# Autodesk Inventor assembly: Sensor_Test
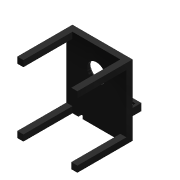
[picture p0: Inventor's stored thumbnail of the model, 180x180]
Saved by Autodesk Inventor 2020 (Build 240168000, 168)
## iProperties
Created: 2022-02-19
Part Number: Sensor_Test
Document SubType Name: Assembly
Designer: Julian Uhl
Author: Julian Uhl
## Documents named in this file (3)
- C:\Schule\Eier-Inventor\Sensor_Test.iam
- C:\Schule\Eier-Inventor\Senso_Halter.ipt
- C:\Schule\Eier-Inventor\Sensor_Dummy.ipt
## Components (2 placed, 2 different names)
1. Senso_Halter:1 — Passend:1, Passend:2, Passend:3
2. Sensor_Dummy:1 — Passend:1, Passend:2, Passend:3
## Relationships (3: Mate 3)
- Passend:1 [Mate]: Senso_Halter:1 ↔ Sensor_Dummy:1
- Passend:2 [Mate]: Senso_Halter:1 ↔ Sensor_Dummy:1
- Passend:3 [Mate]: Senso_Halter:1 ↔ Sensor_Dummy:1
